# Autodesk Inventor assembly: TestRig
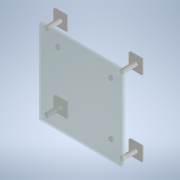
[picture p0: Inventor's stored thumbnail of the model, 180x180]
Saved by Autodesk Inventor 2020.3 (Build 243373010, 373A)
## iProperties
Created: 2020-10-30
Part Number: TestRig
Document SubType Name: Assembly
Designer: Naude Conradie
Author: Naude Conradie
## Documents named in this file (5)
- C:\Users\Naude Conradie\Desktop\Repository\Masters-Project\Models\Inventor\Testing Rig\TestRig.iam
- C:\Users\Naude Conradie\Desktop\Repository\Masters-Project\Models\Inventor\Testing Rig\Plate.ipt
- C:\Users\Naude Conradie\Desktop\Repository\Masters-Project\Models\Inventor\Testing Rig\PlateHoled.ipt
- C:\Users\Naude Conradie\Desktop\Repository\Masters-Project\Models\Inventor\Testing Rig\Plug.ipt
- C:\Users\Naude Conradie\Desktop\Repository\Masters-Project\Models\Inventor\Testing Rig\Leg.ipt
## Components (10 placed, 4 different names)
1. Plate:1 — Mate:4, Flush:3, Mate:22
2. PlateHoled:1 — Mate:4, Flush:3, Mate:6, Mate:7, Mate:8, Mate:9, Mate:10, Mate:11, Mate:12, Mate:13, Mate:14, Mate:15, Mate:16, Mate:17, Mate:18, Mate:19, Mate:20, Mate:21, Angle:1, Angle:2, Angle:3, Angle:4, Mate:22
3. Plug:1 — Mate:10, Mate:11
4. Plug:2 — Mate:12, Mate:13
5. Plug:3 — Mate:8, Mate:9
6. Plug:4 — Mate:6, Mate:7
7. Leg:1 — Mate:14, Mate:18, Angle:1
8. Leg:2 — Mate:15, Mate:19, Angle:2
9. Leg:3 — Mate:16, Mate:20, Angle:3
10. Leg:4 — Mate:17, Mate:21, Angle:4
## Relationships (23: Mate 18, Angle 4, Flush 1)
- Mate:4: Plate:1 ↔ PlateHoled:1
- Flush:3: Plate:1 ↔ PlateHoled:1
- Mate:6: PlateHoled:1 ↔ Plug:4
- Mate:7: PlateHoled:1 ↔ Plug:4
- Mate:8: PlateHoled:1 ↔ Plug:3
- Mate:9: PlateHoled:1 ↔ Plug:3
- Mate:10: PlateHoled:1 ↔ Plug:1
- Mate:11: PlateHoled:1 ↔ Plug:1
- Mate:12: PlateHoled:1 ↔ Plug:2
- Mate:13: PlateHoled:1 ↔ Plug:2
- Mate:14: PlateHoled:1 ↔ Leg:1
- Mate:15: PlateHoled:1 ↔ Leg:2
- Mate:16: PlateHoled:1 ↔ Leg:3
- Mate:17: PlateHoled:1 ↔ Leg:4
- Mate:18: PlateHoled:1 ↔ Leg:1
- Mate:19: PlateHoled:1 ↔ Leg:2
- Mate:20: PlateHoled:1 ↔ Leg:3
- Mate:21: PlateHoled:1 ↔ Leg:4
- Angle:1 (0 deg): PlateHoled:1 ↔ Leg:1
- Angle:2 (0 deg): PlateHoled:1 ↔ Leg:2
- Angle:3 (0 deg): PlateHoled:1 ↔ Leg:3
- Angle:4 (0 deg): PlateHoled:1 ↔ Leg:4
- Mate:22 (2 mm): Plate:1 ↔ PlateHoled:1
